# Autodesk Inventor assembly: Assembly1
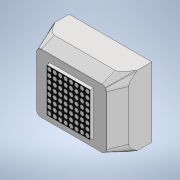
[picture p0: Inventor's stored thumbnail of the model, 180x180]
Saved by Autodesk Inventor 2021 (Build 250183000, 183)
## iProperties
Created: 2023-04-01
Part Number: Assembly1
Document SubType Name: Assembly
Designer: stepa
Author: stepa
## Documents named in this file (8)
- C:\Documents\FEL\1.r\VPP1\3dmodel\Assembly1.iam
- C:\Documents\FEL\1.r\VPP1\3dmodel\Part1.ipt
- C:\Documents\FEL\1.r\VPP1\3dmodel\Part2.ipt
- C:\Documents\FEL\1.r\VPP1\3dmodel\Part4.ipt
- C:\Documents\FEL\1.r\VPP1\3dmodel\Part5.ipt
- C:\Documents\FEL\1.r\VPP1\3dmodel\Part3.ipt
- C:\Documents\FEL\1.r\VPP1\3dmodel\Part6.ipt
- C:\Documents\FEL\1.r\VPP1\3dmodel\body.ipt
## Components (10 placed, 7 different names)
1. Part1:1 — Mate:1, Mate:2, Angle:1, Mate:3, Mate:4, Mate:5, Mate:6, Mate:7, Mate:8, Angle:2, Mate:11
2. Part2:1 — Mate:1
3. Part4:1 — Mate:2, Angle:1
4. Part5:1 — Mate:4
5. Part4:2 — Mate:3
6. Part3:1 — Mate:5
7. Part4:3 — Mate:6
8. Part4:4 — Mate:7
9. Part6:1 — Mate:8, Angle:2, Mate:9, Mate:10
10. body:1 — Mate:9, Mate:10, Mate:11
## Relationships (13: Mate 11, Angle 2)
- Mate:1: Part1:1 ↔ Part2:1
- Mate:2: Part1:1 ↔ Part4:1
- Angle:1 (0 deg): Part1:1 ↔ Part4:1
- Mate:3: Part1:1 ↔ Part4:2
- Mate:4: Part1:1 ↔ Part5:1
- Mate:5: Part1:1 ↔ Part3:1
- Mate:6: Part1:1 ↔ Part4:3
- Mate:7: Part1:1 ↔ Part4:4
- Mate:8: Part1:1 ↔ Part6:1
- Angle:2 (0 deg): Part1:1 ↔ Part6:1
- Mate:9: Part6:1 ↔ body:1
- Mate:10: Part6:1 ↔ body:1
- Mate:11: Part1:1 ↔ body:1
